# Autodesk Inventor assembly: Assembly_Square
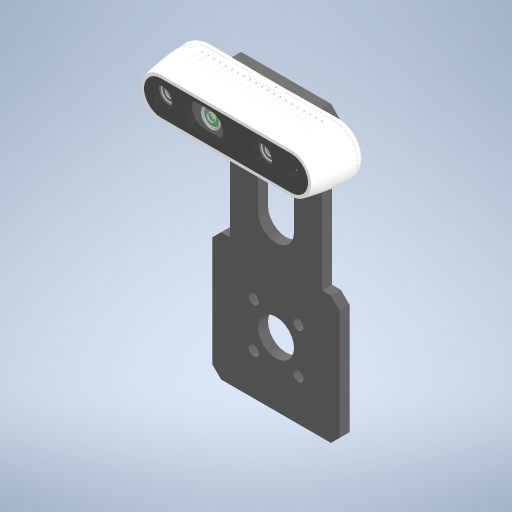
[picture p0: Inventor's stored thumbnail of the model, 512x512]
Saved by Autodesk Inventor 2023 (Build 270158000, 158)
## iProperties
Created: 2022-09-08
Part Number: Assembly_Square
Document SubType Name: Assembly
Designer: romanp
Author: romanp
## Documents named in this file (3)
- C:\Users\romanp\Downloads\RealSense_D435i_+_Holder\pag\Type_1\Assembly_Square.iam
- C:\Users\romanp\Downloads\RealSense_D435i_+_Holder\STEP\IntelRealsense_D435.ipt
- C:\Users\romanp\Downloads\RealSense_D435i_+_Holder\STEP\Part_Type_1_Black.ipt
## Components (2 placed, 2 different names)
1. Part_Type_1_Black:1 — Insert:1, Insert:2
2. IntelRealsense_D435:1 — Insert:1, Insert:2
## Relationships (2: Insert 2)
- Insert:1: Part_Type_1_Black:1 ↔ IntelRealsense_D435:1
- Insert:2: Part_Type_1_Black:1 ↔ IntelRealsense_D435:1
